# Autodesk Inventor assembly: Shock Body
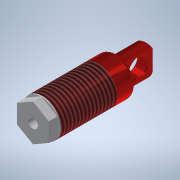
[picture p0: Inventor's stored thumbnail of the model, 180x180]
Saved by Autodesk Inventor 2022.3 (Build 263350000, 350)
## iProperties
Created: 2019-12-02
Part Number: Shock Body
Document SubType Name: Assembly
Designer: Jopa
Author: Jopa
## Documents named in this file (3)
- D:\Luis\Desktop\ESPOL\9 semestre\Itinerario\PIEZAS\PX9200-18_Front-Rear_Shock_Absorber\Shock Body\Shock Body.iam
- D:\Luis\Desktop\ESPOL\9 semestre\Itinerario\PIEZAS\PX9200-18_Front-Rear_Shock_Absorber\Shock Body\Shock Body 1.3 Length.ipt
- D:\Luis\Desktop\ESPOL\9 semestre\Itinerario\PIEZAS\PX9200-18_Front-Rear_Shock_Absorber\Shock Body\Shock Cartridge\Shock Cartridge.iam
## Components (2 placed, 2 different names)
1. Shock Body 1.3 Length:1 — Mate:1, Mate:2, Angle:1
2. Shock Cartridge:1 [sub-assembly] — Mate:1, Mate:2, Angle:1
## Relationships (3: Mate 2, Angle 1)
- Mate:1: Shock Body 1.3 Length:1 ↔ Shock Cartridge:1
- Mate:2: Shock Body 1.3 Length:1 ↔ Shock Cartridge:1
- Angle:1 (0 deg): Shock Body 1.3 Length:1 ↔ Shock Cartridge:1
